# Autodesk Inventor assembly: 15102898-16-A-0000
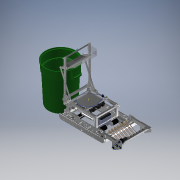
[picture p0: Inventor's stored thumbnail of the model, 180x180]
Saved by Autodesk Inventor 2017 (Build 210142000, 142)
## iProperties
Created: 2016-09-11
Part Number: 15102898-16-A-0000
Document SubType Name: Assembly
Designer: gus
Mass: 27886.1 g
Surface Area: 91797.7 cm^2
Volume: 21610.5 cm^3
Density: 1.2904 g/cm^3
Author: gus
## Documents named in this file (13)
- \\Mac\Home\Desktop\bunnybots 2016\15102898-16-Bunnybot-CAD\Bunnybot-To_be_renamed\15102898-16-A-0000\15102898-16-A-0000.iam
- \\Mac\Home\Desktop\bunnybots 2016\15102898-16-Bunnybot-CAD\Bunnybot-To_be_renamed\15102898-16-A-0000\15102898-16-A-0100\15102898-16-A-0100.iam
- \\Mac\Home\Desktop\bunnybots 2016\15102898-16-Bunnybot-CAD\Bunnybot-To_be_renamed\15102898-16-A-0000\15102898-16-A-0200\15102898-16-A-0200.iam
- \\Mac\Home\Desktop\bunnybots 2016\15102898-16-Bunnybot-CAD\Bunnybot-To_be_renamed\15102898-16-A-0000\15102898-16-A-0300\15102898-16-A-0300.iam
- \\Mac\Home\Desktop\bunnybots 2016\15102898-16-Bunnybot-CAD\Bunnybot-To_be_renamed\15102898-16-A-0000\recycling bin\RECYCLING_CAN.ipt
- \\Mac\Home\Desktop\bunnybots 2016\15102898-16-Bunnybot-CAD\Bunnybot-To_be_renamed\15102898-16-A-0000\15102898-16-A-0400\15102898-16-A-0400.iam
- \\Mac\Home\Desktop\bunnybots 2016\15102898-16-Bunnybot-CAD\Bunnybot-To_be_renamed\15102898-16-A-0000\15102898-16-A-0300\15102898-16-P-0306.ipt
- \\Mac\Home\Desktop\bunnybots 2016\15102898-16-Bunnybot-CAD\Bunnybot-To_be_renamed\15102898-16-A-0000\15102898-16-A-0300\15102898-16-P-0306_MIR.ipt
- \\Mac\Home\Desktop\bunnybots 2016\15102898-16-Bunnybot-CAD\Bunnybot-To_be_renamed\15102898-16-A-0000\15102898-16-A-0600\Turret ASM.iam
- \\Mac\Home\Desktop\bunnybots 2016\15102898-16-Bunnybot-CAD\Bunnybot-To_be_renamed\15102898-16-A-0000\Pneumatics\Pneu_Tank_AVT-PP-35.ipt
- \\Mac\Home\Desktop\bunnybots 2016\15102898-16-Bunnybot-CAD\Bunnybot-To_be_renamed\15102898-16-A-0000\Pneumatics\Run01\15102898-16-A-0000.Tube and Pipe Runs.iam
- \\Mac\Home\Desktop\bunnybots 2016\15102898-16-Bunnybot-CAD\Bunnybot-To_be_renamed\15102898-16-A-0000\15102898-16-A-0700\1510-2898-A-0700.iam
- \\Mac\Home\Desktop\bunnybots 2016\15102898-16-Bunnybot-CAD\Bunnybot-To_be_renamed\15102898-16-A-0000\15102898-16-A-0800\15102898-16-A-0800.iam
## Components (15 placed, 12 different names)
1. 15102898-16-A-0100:1 [sub-assembly] — Mate:1, Mate:3, Mate:4, Flush:1, Mate:5, Flush:2, Mate:6, Flush:3, Mate:7, Mate:8, Flush:5, Mate:12, Mate:13, Mate:14, Flush:16, Mate:15
2. 15102898-16-A-0200:1 [sub-assembly] — Mate:1, Mate:3, Mate:4, Mate:9, Flush:11, Flush:12, Tangent:8
3. 15102898-16-A-0300:2 [sub-assembly] — Rotational:1
4. RECYCLING_CAN:1
5. 15102898-16-A-0400:1 [sub-assembly] — Mate:5, Flush:2, Mate:6
6. 15102898-16-P-0306:1 — Flush:3, Mate:7, Rotational:1, Mate:8, Flush:4, Flush:6, Flush:17
7. 15102898-16-P-0306_MIR:1 — Flush:4, Flush:5, Flush:6
8. Turret ASM:1 [sub-assembly] — Mate:9, Flush:11, Flush:12, Tangent:1, Tangent:2, Tangent:3, Tangent:4, Mate:10
9. Pneu_Tank_AVT-PP-35:1 — Tangent:1, Tangent:6, Tangent:7, Flush:13, Flush:14
10. Pneu_Tank_AVT-PP-35:2 — Tangent:2, Tangent:5, Tangent:6, Flush:14, Flush:15
11. Pneu_Tank_AVT-PP-35:3 — Tangent:4, Tangent:5, Flush:15
12. Pneu_Tank_AVT-PP-35:4 — Tangent:3, Tangent:7, Flush:13, Mate:10, Tangent:8
13. 15102898-16-A-0000.Tube and Pipe Runs:1 [sub-assembly]
14. 1510-2898-A-0700:1 [sub-assembly] — Mate:12, Mate:13, Mate:14
15. 15102898-16-A-0800:1 [sub-assembly] — Flush:16, Mate:15, Flush:17
## Relationships (35: Mate 13, Flush 13, Tangent 8, RevoluteJoint 1)
- Mate:1: 15102898-16-A-0100:1 ↔ 15102898-16-A-0200:1
- Mate:3 (34.925 mm): 15102898-16-A-0100:1 ↔ 15102898-16-A-0200:1
- Mate:4 (3.175 mm): 15102898-16-A-0100:1 ↔ 15102898-16-A-0200:1
- Flush:1 (-291.973 mm): 15102898-16-A-0100:1
- Mate:5: 15102898-16-A-0100:1 ↔ 15102898-16-A-0400:1
- Flush:2: 15102898-16-A-0100:1 ↔ 15102898-16-A-0400:1
- Mate:6: 15102898-16-A-0100:1 ↔ 15102898-16-A-0400:1
- Flush:3: 15102898-16-A-0100:1 ↔ 15102898-16-P-0306:1
- Mate:7: 15102898-16-A-0100:1 ↔ 15102898-16-P-0306:1
- Rotational:1 [RevoluteJoint]: 15102898-16-A-0300:2 ↔ 15102898-16-P-0306:1
- Mate:8: 15102898-16-A-0100:1 ↔ 15102898-16-P-0306:1
- Flush:4: 15102898-16-P-0306:1 ↔ 15102898-16-P-0306_MIR:1
- Flush:5: 15102898-16-A-0100:1 ↔ 15102898-16-P-0306_MIR:1
- Flush:6: 15102898-16-P-0306:1 ↔ 15102898-16-P-0306_MIR:1
- Mate:9: 15102898-16-A-0200:1 ↔ Turret ASM:1
- Flush:11: 15102898-16-A-0200:1 ↔ Turret ASM:1
- Flush:12 (127 mm): 15102898-16-A-0200:1 ↔ Turret ASM:1
- Tangent:1: Turret ASM:1 ↔ Pneu_Tank_AVT-PP-35:1
- Tangent:2: Turret ASM:1 ↔ Pneu_Tank_AVT-PP-35:2
- Tangent:3: Turret ASM:1 ↔ Pneu_Tank_AVT-PP-35:4
- Tangent:4: Turret ASM:1 ↔ Pneu_Tank_AVT-PP-35:3
- Tangent:5: Pneu_Tank_AVT-PP-35:2 ↔ Pneu_Tank_AVT-PP-35:3
- Tangent:6 (25.4 mm): Pneu_Tank_AVT-PP-35:1 ↔ Pneu_Tank_AVT-PP-35:2
- Tangent:7: Pneu_Tank_AVT-PP-35:1 ↔ Pneu_Tank_AVT-PP-35:4
- Flush:13: Pneu_Tank_AVT-PP-35:1 ↔ Pneu_Tank_AVT-PP-35:4
- Flush:14: Pneu_Tank_AVT-PP-35:1 ↔ Pneu_Tank_AVT-PP-35:2
- Flush:15: Pneu_Tank_AVT-PP-35:2 ↔ Pneu_Tank_AVT-PP-35:3
- Mate:10: Turret ASM:1 ↔ Pneu_Tank_AVT-PP-35:4
- Tangent:8: 15102898-16-A-0200:1 ↔ Pneu_Tank_AVT-PP-35:4
- Mate:12: 15102898-16-A-0100:1 ↔ 1510-2898-A-0700:1
- Mate:13: 15102898-16-A-0100:1 ↔ 1510-2898-A-0700:1
- Mate:14: 15102898-16-A-0100:1 ↔ 1510-2898-A-0700:1
- Flush:16: 15102898-16-A-0100:1 ↔ 15102898-16-A-0800:1
- Mate:15: 15102898-16-A-0100:1 ↔ 15102898-16-A-0800:1
- Flush:17 (-3.175 mm): 15102898-16-P-0306:1 ↔ 15102898-16-A-0800:1
